# Autodesk Inventor assembly: 6ep13111sh12
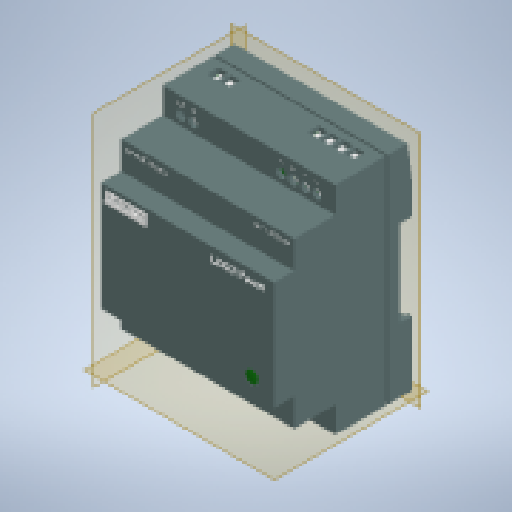
[picture p0: Inventor's stored thumbnail of the model, 512x512]
Saved by Autodesk Inventor 2025.2 (Build 292293000, 293)
## iProperties
Created: 2020-01-23
Part Number: 6ep13111sh12
Checked By: TraceParts S.A.
Catalog Web Link: www.traceparts.com
Document SubType Name: Assembly
Designer: TraceParts
Company: TraceParts S.A.
REFERENCE: 6EP13111SH12
DESIGN: Logo! power 5V stabilized power supply input: 100-240V AC output: 5V DC/6.3A
SUPPLIER: SIEMENS
TraceParts.PartNumber: 90-02042019-042683
TraceParts.PartTitle: Continuous current supply
TraceParts.InstanceId: 90-02042019-0426831062XH0K9RCMD6AYA3G7LUMMH
TraceParts.PartStatus: Published
TraceParts.PartVersion: 1.0.0
TRACEPARTS: TRACEPARTS
TraceParts.PartLanguage: en
TraceParts.ClassPath: SIEMENS_AUTOMATION:90-02042019-042683
Author: TraceParts
## Documents named in this file (5)
- C:\Users\lucas\OneDrive\Documentos\Documentos\Gustavo\Mozangao\Projeto Base (5140)\Q.E - Braço Robotico\Fonte de Alimentacao\f_alimentacao_230ac-5vdc_0001_001.iam
- C:\Users\lucas\OneDrive\Documentos\Documentos\Gustavo\Mozangao\Projeto Base (5140)\Q.E - Braço Robotico\Fonte de Alimentacao\f_alimentacao_230ac-5vdc_0002_001.ipt
- C:\Users\lucas\OneDrive\Documentos\Documentos\Gustavo\Mozangao\Projeto Base (5140)\Q.E - Braço Robotico\Fonte de Alimentacao\f_alimentacao_230ac-5vdc_0003_001.ipt
- C:\Users\lucas\OneDrive\Documentos\Documentos\Gustavo\Mozangao\Projeto Base (5140)\Q.E - Braço Robotico\Fonte de Alimentacao\f_alimentacao_230ac-5vdc_0004_001.ipt
- C:\Users\lucas\OneDrive\Documentos\Documentos\Gustavo\Mozangao\Projeto Base (5140)\Q.E - Braço Robotico\Fonte de Alimentacao\f_alimentacao_230ac-5vdc_0005_001.ipt
## Components (4 placed, 4 different names)
1. f_alimentacao_230ac-5vdc_0002_001:1
2. f_alimentacao_230ac-5vdc_0003_001:1
3. f_alimentacao_230ac-5vdc_0004_001:1
4. f_alimentacao_230ac-5vdc_0005_001:1 — Alinhado:1
## Relationships (1: Flush 1)
- Alinhado:1 [Flush] (-36 mm): f_alimentacao_230ac-5vdc_0005_001:1
